# Autodesk Inventor assembly: Body-40x
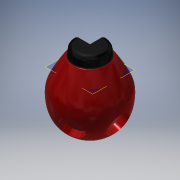
[picture p0: Inventor's stored thumbnail of the model, 180x180]
Saved by Autodesk Inventor 2018 (Build 220112000, 112)
## iProperties
Created: 2017-08-21
Part Number: Body-40x
Material: Generisch
Document SubType Name: Assembly
Designer: JochenAlt
Author: JochenAlt
## Documents named in this file (9)
- D:\Projects\Manfred\design\cad\Inventor\Body-40x.iam
- D:\Projects\Manfred\design\cad\Inventor\Body-40x.ipt
- D:\Projects\Manfred\design\cad\Inventor\PCB Slamtec RPLidar A2.ipt
- D:\Projects\Manfred\design\cad\Inventor\RPLidar A2.ipt
- D:\Projects\Manfred\design\cad\Inventor\Battery Pack.iam
- D:\Projects\Manfred\design\cad\Inventor\BNO055.ipt
- D:\Projects\Manfred\design\cad\Inventor\ODroid Holder-40x.ipt
- D:\Projects\Manfred\design\cad\Inventor\Lidar-Holder-40x.ipt
- D:\Projects\Manfred\design\cad\Inventor\ODroid C2\ODroid C2.iam
## Components (8 placed, 8 different names)
1. Body-40x:1 — Passend:35, Winkel:2, Passend:37, Passend:39
2. RPLidar A2:1 — Passend:41, Passend:42
3. PCB Slamtec RPLidar A2:1 — Passend:53, Passend:54
4. BNO055:1 — Passend:50, Passend:51
5. Battery Pack:1 [sub-assembly] — Passend:38, Passend:39, Passend:40, Winkel:5
6. ODroid Holder-40x:1 — Passend:33, Passend:35, Winkel:2, Passend:36, Passend:37, Passend:38, Passend:40, Passend:47, Winkel:4, Winkel:5, Passend:55
7. Lidar-Holder-40x:1 — Passend:41, Passend:42, Passend:47, Passend:50, Passend:51, Winkel:4, Passend:53, Passend:54, Passend:55
8. ODroid C2:1 [sub-assembly] — Passend:33, Passend:36
## Relationships (18: Mate 15, Angle 3)
- Passend:33 [Mate]: ODroid Holder-40x:1 ↔ ODroid C2:1
- Passend:35 [Mate]: Body-40x:1 ↔ ODroid Holder-40x:1
- Winkel:2 [Angle] (180 deg): Body-40x:1 ↔ ODroid Holder-40x:1
- Passend:36 [Mate]: ODroid Holder-40x:1 ↔ ODroid C2:1
- Passend:37 [Mate]: Body-40x:1 ↔ ODroid Holder-40x:1
- Passend:38 [Mate]: Battery Pack:1 ↔ ODroid Holder-40x:1
- Passend:39 [Mate]: Body-40x:1 ↔ Battery Pack:1
- Passend:40 [Mate]: Battery Pack:1 ↔ ODroid Holder-40x:1
- Passend:41 [Mate]: RPLidar A2:1 ↔ Lidar-Holder-40x:1
- Passend:42 [Mate]: RPLidar A2:1 ↔ Lidar-Holder-40x:1
- Passend:47 [Mate]: ODroid Holder-40x:1 ↔ Lidar-Holder-40x:1
- Passend:50 [Mate]: BNO055:1 ↔ Lidar-Holder-40x:1
- Passend:51 [Mate]: BNO055:1 ↔ Lidar-Holder-40x:1
- Winkel:4 [Angle] (180 deg): ODroid Holder-40x:1 ↔ Lidar-Holder-40x:1
- Winkel:5 [Angle] (0 deg): Battery Pack:1 ↔ ODroid Holder-40x:1
- Passend:53 [Mate]: PCB Slamtec RPLidar A2:1 ↔ Lidar-Holder-40x:1
- Passend:54 [Mate]: PCB Slamtec RPLidar A2:1 ↔ Lidar-Holder-40x:1
- Passend:55 [Mate] (0.2 mm): ODroid Holder-40x:1 ↔ Lidar-Holder-40x:1
